# Autodesk Inventor assembly: Naveeassembly.ipt
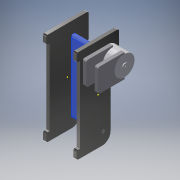
[picture p0: Inventor's stored thumbnail of the model, 180x180]
Saved by Autodesk Inventor 2019 (Build 230136000, 136)
## iProperties
Created: 2020-03-06
Part Number: Naveeassembly.ipt
Document SubType Name: Assembly
Designer: HP
Author: HP
## Documents named in this file (8)
- C:\Users\HP\OneDrive\Documents\Inventor\Content Center Files\Naveeassembly.ipt.iam
- C:\Users\HP\OneDrive\Documents\Inventor\Content Center Files\R2019\1belt.ipt
- C:\Users\HP\OneDrive\Documents\Inventor\Content Center Files\R2019\1shaft.ipt
- C:\Users\HP\OneDrive\Documents\Inventor\Content Center Files\R2019\11side.ipt
- C:\Users\HP\OneDrive\Documents\Inventor\Content Center Files\Assemble\Motor DC.ipt
- C:\Users\HP\OneDrive\Documents\Inventor\Content Center Files\R2019\2stand.ipt
- C:\Users\HP\OneDrive\Documents\Inventor\Content Center Files\Assemble\car_assembly.iam
- C:\Users\HP\OneDrive\Documents\Inventor\Content Center Files\R2019\1servo.ipt
## Components (11 placed, 7 different names)
1. 1belt:1 — Mate:1, Mate:2, Mate:7
2. 1shaft:1 — Mate:1, Mate:3, Mate:4, Flush:1, Flush:4, Mate:8
3. 1shaft:2 — Mate:2, Mate:5, Mate:6, Flush:2, Flush:3
4. 11side:1 — Mate:4, Mate:5, Flush:1, Mate:7, Flush:3, Rigid:1
5. 11side:2 — Mate:3, Mate:6, Flush:2, Flush:4
6. Motor DC:1 — Mate:8, Rigid:1, Rotational:1, Flush:5, Mate:9
7. 2stand:1 — Rotational:1, Flush:5, Rigid:2
8. 2stand:2 — Mate:9, Rigid:2
9. car_assembly:1 [sub-assembly]
10. 1servo:1
11. 1servo:2
## Relationships (17: Mate 9, Flush 5, WeldJoint 2, RevoluteJoint 1)
- Mate:1: 1belt:1 ↔ 1shaft:1
- Mate:2: 1belt:1 ↔ 1shaft:2
- Mate:3: 1shaft:1 ↔ 11side:2
- Mate:4: 1shaft:1 ↔ 11side:1
- Mate:5: 1shaft:2 ↔ 11side:1
- Mate:6: 1shaft:2 ↔ 11side:2
- Flush:1: 1shaft:1 ↔ 11side:1
- Flush:2: 1shaft:2 ↔ 11side:2
- Mate:7 (5 mm): 1belt:1 ↔ 11side:1
- Flush:3: 1shaft:2 ↔ 11side:1
- Flush:4: 1shaft:1 ↔ 11side:2
- Mate:8: 1shaft:1 ↔ Motor DC:1
- Rigid:1 [WeldJoint]: 11side:1 ↔ Motor DC:1
- Rotational:1 [RevoluteJoint]: Motor DC:1 ↔ 2stand:1
- Flush:5: Motor DC:1 ↔ 2stand:1
- Mate:9: Motor DC:1 ↔ 2stand:2
- Rigid:2 [WeldJoint] (50 mm): 2stand:1 ↔ 2stand:2
